# Autodesk Inventor assembly: Joist_With_Length_144_Inches
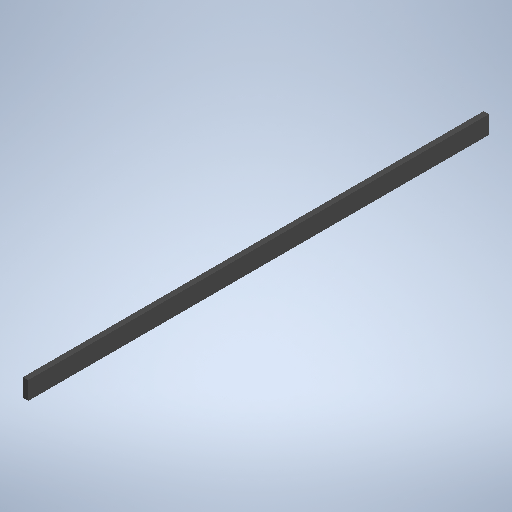
[picture p0: Inventor's stored thumbnail of the model, 512x512]
Saved by Autodesk Inventor 2025 (Build 290162010, 162A)
## iProperties
Created: 2024-09-15
Part Number: Joist_With_Length_144_Inches
Document SubType Name: Assembly
Designer: Tom
Author: Tom
## Documents named in this file (4)
- C:\Users\Tom\Documents\Inventor\Mobility\Additional_Building\Joist_With_Length_144_Inches.iam
- C:\Users\Tom\Documents\Inventor\Mobility\Additional_Building\Joist_With_Length_144_Inches.ipt
- C:\Users\Tom\Documents\Inventor\Mobility\Additional_Building\Tube_Of_Underlayment_For_Joist_With_Length_144_Inches.ipt
- C:\Users\Tom\Documents\Inventor\Mobility\Additional_Building\Rectangle_Of_Underlayment_For_Joist.ipt
## Components (4 placed, 3 different names)
1. Joist_With_Length_144_Inches:1 — Mate:1, Flush:1, Flush:2, Mate:2, Flush:3, Flush:4, Mate:3, Mate:4
2. Tube_Of_Underlayment_For_Joist_With_Length_144_Inches:1 — Mate:3, Mate:4, Flush:5
3. Rectangle_Of_Underlayment_For_Joist:1 — Mate:1, Flush:1, Flush:2, Flush:5
4. Rectangle_Of_Underlayment_For_Joist:2 — Mate:2, Flush:3, Flush:4
## Relationships (9: Flush 5, Mate 4)
- Mate:1: Joist_With_Length_144_Inches:1 ↔ Rectangle_Of_Underlayment_For_Joist:1
- Flush:1: Joist_With_Length_144_Inches:1 ↔ Rectangle_Of_Underlayment_For_Joist:1
- Flush:2: Joist_With_Length_144_Inches:1 ↔ Rectangle_Of_Underlayment_For_Joist:1
- Mate:2: Joist_With_Length_144_Inches:1 ↔ Rectangle_Of_Underlayment_For_Joist:2
- Flush:3: Joist_With_Length_144_Inches:1 ↔ Rectangle_Of_Underlayment_For_Joist:2
- Flush:4: Joist_With_Length_144_Inches:1 ↔ Rectangle_Of_Underlayment_For_Joist:2
- Mate:3: Joist_With_Length_144_Inches:1 ↔ Tube_Of_Underlayment_For_Joist_With_Length_144_Inches:1
- Mate:4: Joist_With_Length_144_Inches:1 ↔ Tube_Of_Underlayment_For_Joist_With_Length_144_Inches:1
- Flush:5: Tube_Of_Underlayment_For_Joist_With_Length_144_Inches:1 ↔ Rectangle_Of_Underlayment_For_Joist:1
